# Autodesk Inventor assembly: magnet_ring_assembly
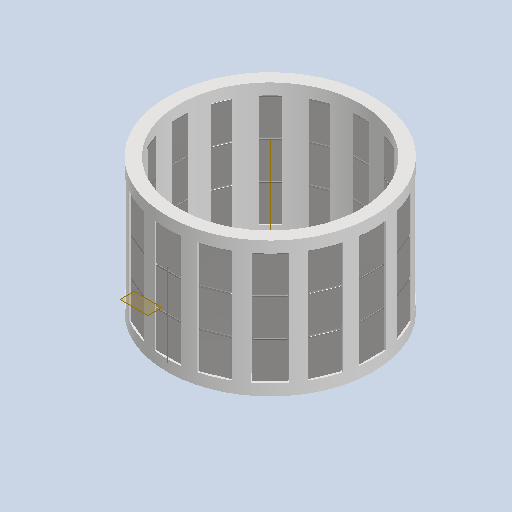
[picture p0: Inventor's stored thumbnail of the model, 512x512]
Saved by Autodesk Inventor 2025 (Build 290162000, 162)
## iProperties
Created: 2026-08-03
Part Number: magnet_ring_assembly
Document SubType Name: Assembly
Designer: zzapa
Author: zzapa
## Documents named in this file (3)
- C:\Users\zzapa\Desktop\Projekty\elektronika\engine-project\model\assemblies\magnet_ring_assembly.iam
- C:\Users\zzapa\Desktop\Projekty\elektronika\engine-project\model\parts\magnet_ring.ipt
- C:\Users\zzapa\Desktop\Projekty\elektronika\engine-project\model\parts\stator_magnet.ipt
## Components (49 placed, 2 different names)
1. magnet_ring:1 — Zestawiające:1, Zestawiające:2, Kątowe:1, Zestawiające:6, Równoległe:5, Zestawiające:7
2. stator_magnet:1 — Zestawiające:3, Równoległe:1, Równoległe:2, Zestawiające:6, Symetria:1, Symetria:2
3. stator_magnet:2 — Zestawiające:4, Równoległe:3, Równoległe:4, Symetria:1
4. stator_magnet:3 — Zestawiające:3, Równoległe:1, Zestawiające:4, Równoległe:2, Równoległe:3, Równoległe:4, Zestawiające:7, Symetria:2
5. stator_magnet:4
6. stator_magnet:5
7. stator_magnet:6
8. stator_magnet:7
9. stator_magnet:8
10. stator_magnet:9
11. stator_magnet:10
12. stator_magnet:11
13. stator_magnet:12
14. stator_magnet:13
15. stator_magnet:14
16. stator_magnet:15
17. stator_magnet:16
18. stator_magnet:17
19. stator_magnet:18
20. stator_magnet:19
21. stator_magnet:20
22. stator_magnet:21
23. stator_magnet:22
24. stator_magnet:23
25. stator_magnet:24
26. stator_magnet:25
27. stator_magnet:26
28. stator_magnet:27
29. stator_magnet:28
30. stator_magnet:29
31. stator_magnet:30
32. stator_magnet:31
33. stator_magnet:32
34. stator_magnet:33
35. stator_magnet:34
36. stator_magnet:35
37. stator_magnet:36
38. stator_magnet:37
39. stator_magnet:38
40. stator_magnet:39
41. stator_magnet:40
42. stator_magnet:41
43. stator_magnet:42
44. stator_magnet:43
45. stator_magnet:44
46. stator_magnet:45
47. stator_magnet:46
48. stator_magnet:47
49. stator_magnet:48
## Component patterns: (16 elements, first: stator_magnet:1 + stator_magnet:2 + stator_magnet:3)
## Relationships (15: Mate 6, Flush 6, Symmetry 2, Angle 1)
- Zestawiające:1 [Mate]: magnet_ring:1
- Zestawiające:2 [Mate]: magnet_ring:1
- Kątowe:1 [Angle] (0 deg): magnet_ring:1
- Zestawiające:3 [Mate]: stator_magnet:1 ↔ stator_magnet:3
- Równoległe:1 [Flush]: stator_magnet:1 ↔ stator_magnet:3
- Zestawiające:4 [Mate]: stator_magnet:2 ↔ stator_magnet:3
- Równoległe:2 [Flush]: stator_magnet:1 ↔ stator_magnet:3
- Równoległe:3 [Flush]: stator_magnet:2 ↔ stator_magnet:3
- Równoległe:4 [Flush]: stator_magnet:2 ↔ stator_magnet:3
- Zestawiające:6 [Mate]: magnet_ring:1 ↔ stator_magnet:1
- Symetria:1 [Symmetry]: stator_magnet:1 ↔ stator_magnet:2
- Równoległe:5 [Flush]: magnet_ring:1
- Zestawiające:7 [Mate]: magnet_ring:1 ↔ stator_magnet:3
- Symetria:2 [Symmetry]: stator_magnet:1 ↔ stator_magnet:3
- Równoległe:6 [Flush]
